# Autodesk Inventor assembly: ScaraNema
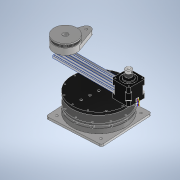
[picture p0: Inventor's stored thumbnail of the model, 180x180]
Saved by Autodesk Inventor 2022 (Build 260153000, 153)
## iProperties
Created: 2022-02-16
Part Number: ScaraNema
Document SubType Name: Assembly
Designer: JK
Author: JK
## Documents named in this file (3)
- C:\Users\JK\Documents\Inventor\ScaraNema\ScaraNema.iam
- C:\Users\JK\Documents\Inventor\ScaraNema\Inverse timing belt reducer\Inverse belt reducer.iam
- C:\Users\JK\Documents\Inventor\ScaraNema\elbowassembly.iam
## Components (2 placed, 2 different names)
1. Inverse belt reducer:1 [sub-assembly] — Coincidencia:1
2. elbowassembly:1 [sub-assembly] — Coincidencia:1
## Relationships (1: Mate 1)
- Coincidencia:1 [Mate]: Inverse belt reducer:1 ↔ elbowassembly:1
